# Autodesk Inventor assembly: Assely_Curve_Liner
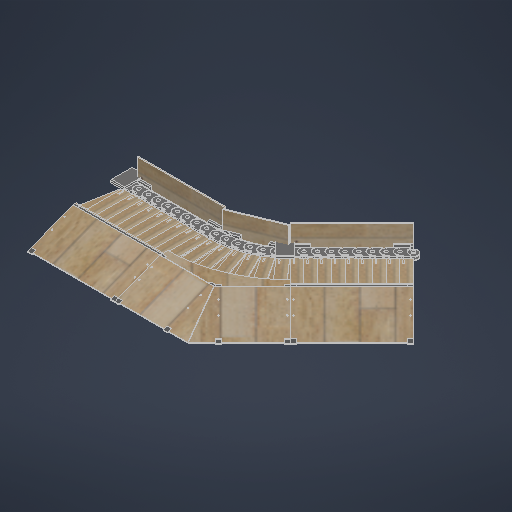
[picture p0: Inventor's stored thumbnail of the model, 512x512]
Saved by Autodesk Inventor 2026.3 (Build 303398000, 398)
## iProperties
Created: 2026-09-07
Part Number: Assely_Curve_Liner
Document SubType Name: Assembly
Designer: takuya
Author: takuya
## Documents named in this file (3)
- D:\model\D2_Conveyor_2026\Assely_Curve_Liner.iam
- D:\model\D2_Conveyor_2026\liniar_module\Assy_linear_module.iam
- D:\model\D2_Conveyor_2026\curve_module\Assy_curve_module.iam
## Components (3 placed, 2 different names)
1. Assy_linear_module:2 [sub-assembly] — メイト:1, フラッシュ:2, フラッシュ:3
2. Assy_linear_module:3 [sub-assembly] — メイト:2, フラッシュ:1, フラッシュ:4
3. Assy_curve_module:1 [sub-assembly] — メイト:1, メイト:2, フラッシュ:1, フラッシュ:2, フラッシュ:3, フラッシュ:4
## Relationships (6: Flush 4, Mate 2)
- メイト:1 [Mate]: Assy_linear_module:2 ↔ Assy_curve_module:1
- メイト:2 [Mate]: Assy_linear_module:3 ↔ Assy_curve_module:1
- フラッシュ:1 [Flush]: Assy_linear_module:3 ↔ Assy_curve_module:1
- フラッシュ:2 [Flush]: Assy_linear_module:2 ↔ Assy_curve_module:1
- フラッシュ:3 [Flush]: Assy_linear_module:2 ↔ Assy_curve_module:1
- フラッシュ:4 [Flush]: Assy_linear_module:3 ↔ Assy_curve_module:1
